# Autodesk Inventor assembly: full
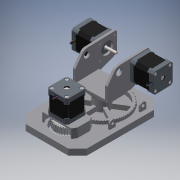
[picture p0: Inventor's stored thumbnail of the model, 180x180]
Saved by Autodesk Inventor 2019 (Build 230136000, 136)
## iProperties
Created: 2019-05-15
Part Number: full
Document SubType Name: Assembly
Designer: Nathan
Author: Nathan
## Documents named in this file (5)
- C:\Users\Nathan\workspace\fbd-brachium\cad\full.iam
- C:\Users\Nathan\workspace\fbd-brachium\cad\shoulder.ipt
- C:\Users\Nathan\workspace\fbd-brachium\cad\nema17.ipt
- C:\Users\Nathan\workspace\fbd-brachium\cad\base.ipt
- C:\Users\Nathan\workspace\fbd-brachium\cad\full\Design Accelerator\Spur Gears1.iam
## Components (6 placed, 4 different names)
1. shoulder:1 — Insert:1, Insert:2, Insert:3, Insert:4, Insert:5
2. nema17:1 — Insert:3, Insert:4
3. nema17:2 — Insert:1, Insert:2
4. base:1 — Insert:5, Insert:6, Insert:7
5. nema17:3 — Insert:6, Insert:7, Mate:1
6. Spur Gears:1 [sub-assembly] — Mate:1
## Relationships (8: Insert 7, Mate 1)
- Insert:1: shoulder:1 ↔ nema17:2
- Insert:2: shoulder:1 ↔ nema17:2
- Insert:3: shoulder:1 ↔ nema17:1
- Insert:4: shoulder:1 ↔ nema17:1
- Insert:5: shoulder:1 ↔ base:1
- Insert:6: base:1 ↔ nema17:3
- Insert:7: base:1 ↔ nema17:3
- Mate:1: nema17:3 ↔ Spur Gears:1
